# Autodesk Inventor assembly: Galvo-Cage-testassembly1
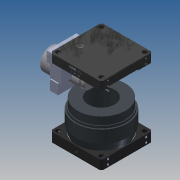
[picture p0: Inventor's stored thumbnail of the model, 180x180]
Saved by Autodesk Inventor 2019 (Build 230136000, 136)
## iProperties
Created: 2019-12-17
Part Number: Galvo-Cage-testassembly1
Document SubType Name: Assembly
Designer: voigt
Author: voigt
## Documents named in this file (7)
- J:\Microscope_Design\CAD_Files\mesoSPIM_design_benchtop_V1\mesoSPIM\excitation_path\Galvo-Cage-testassembly1.iam
- J:\Microscope_Design\CAD_Files\mesoSPIM_design_benchtop_V1\mesoSPIM\excitation_path\components\60mm-blank-cageplate-LCP03M-Nikon-MOD.ipt
- J:\Microscope_Design\CAD_Files\mesoSPIM_design_benchtop_V1\library\Thorlabs\other\F-Mount-AdapterSM2NFM-Step.ipt
- J:\Microscope_Design\CAD_Files\mesoSPIM_design_benchtop_V1\library\Nikon\50mm_1_4G_body_disassembled.ipt
- J:\Microscope_Design\CAD_Files\mesoSPIM_design_benchtop_V1\library\Thorlabs\galvos\GVS411_M.ipt
- J:\Microscope_Design\CAD_Files\mesoSPIM_design_benchtop_V1\library\Thorlabs\galvos\GVS411-galvo-bracket-modified.ipt
- J:\Microscope_Design\CAD_Files\mesoSPIM_design_benchtop_V1\library\Thorlabs\60mm_cage_system\LCP03_M_modified_for_GVS411.ipt
## Components (6 placed, 6 different names)
1. 60mm-blank-cageplate-LCP03M-Nikon-MOD:1 — Mate:1, Mate:2, Mate:3, Angle:1, Mate:13, Mate:14
2. F-Mount-AdapterSM2NFM-Step:1 — Mate:1, Mate:2, Mate:4
3. 50mm_1_4G_body_disassembled:1 — Mate:3, Mate:4, Mate:5, Flush:1, Mate:9
4. GVS411_M:1 — Mate:6, Angle:1, Mate:10, Mate:11, Mate:12
5. GVS411-galvo-bracket-modified:1 — Mate:12, Angle:2, Mate:15
6. LCP03_M_modified_for_GVS411:1 — Mate:13, Mate:14, Mate:15
## Relationships (18: Mate 15, Angle 2, Flush 1)
- Mate:1: 60mm-blank-cageplate-LCP03M-Nikon-MOD:1 ↔ F-Mount-AdapterSM2NFM-Step:1
- Mate:2: 60mm-blank-cageplate-LCP03M-Nikon-MOD:1 ↔ F-Mount-AdapterSM2NFM-Step:1
- Mate:3: 60mm-blank-cageplate-LCP03M-Nikon-MOD:1 ↔ 50mm_1_4G_body_disassembled:1
- Mate:4: F-Mount-AdapterSM2NFM-Step:1 ↔ 50mm_1_4G_body_disassembled:1
- Mate:5: 50mm_1_4G_body_disassembled:1
- Flush:1 (12 mm): 50mm_1_4G_body_disassembled:1
- Mate:6: GVS411_M:1
- Mate:7
- Angle:1 (0 deg): 60mm-blank-cageplate-LCP03M-Nikon-MOD:1 ↔ GVS411_M:1
- Mate:8
- Mate:9: 50mm_1_4G_body_disassembled:1
- Mate:10 (14 mm): GVS411_M:1
- Mate:11: GVS411_M:1
- Mate:12: GVS411_M:1 ↔ GVS411-galvo-bracket-modified:1
- Angle:2 (0 deg): GVS411-galvo-bracket-modified:1
- Mate:13: 60mm-blank-cageplate-LCP03M-Nikon-MOD:1 ↔ LCP03_M_modified_for_GVS411:1
- Mate:14: 60mm-blank-cageplate-LCP03M-Nikon-MOD:1 ↔ LCP03_M_modified_for_GVS411:1
- Mate:15: GVS411-galvo-bracket-modified:1 ↔ LCP03_M_modified_for_GVS411:1
